# Autodesk Inventor assembly: Assembly
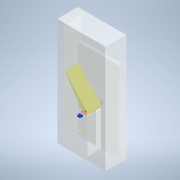
[picture p0: Inventor's stored thumbnail of the model, 180x180]
Saved by Autodesk Inventor 2020 (Build 240168000, 168)
## iProperties
Created: 2019-11-20
Part Number: Assembly
Document SubType Name: Assembly
Designer: camde
Mass: 21034.3 g
Surface Area: 12684.4 cm^2
Volume: 16365.6 cm^3
Density: 1.28527 g/cm^3
Author: camde
## Documents named in this file (5)
- D:\ENGR KC\Bistable Sorter\Assembly.iam
- D:\ENGR KC\Bistable Sorter\ENGR131 KC Design 2.ipt
- D:\ENGR KC\Bistable Sorter\Bistable Rod 2.ipt
- D:\ENGR KC\Bistable Sorter\Bistable Flipper 2.ipt
- D:\ENGR KC\Bistable Sorter\servo motor.ipt
## Components (4 placed, 4 different names)
1. ENGR131 KC Design 2:1 — Mate:4, Mate:5, Mate:8
2. Bistable Rod 2:1 — Mate:1, Mate:3, Mate:4, Mate:6, Mate:7
3. Bistable Flipper 2:1 — Mate:1, Mate:3, Mate:5
4. servo motor:1 — Mate:6, Mate:7, Mate:8
## Relationships (7: Mate 7)
- Mate:1: Bistable Rod 2:1 ↔ Bistable Flipper 2:1
- Mate:3: Bistable Rod 2:1 ↔ Bistable Flipper 2:1
- Mate:4: ENGR131 KC Design 2:1 ↔ Bistable Rod 2:1
- Mate:5: ENGR131 KC Design 2:1 ↔ Bistable Flipper 2:1
- Mate:6: Bistable Rod 2:1 ↔ servo motor:1
- Mate:7: Bistable Rod 2:1 ↔ servo motor:1
- Mate:8: ENGR131 KC Design 2:1 ↔ servo motor:1
